# Autodesk Inventor assembly: Frame
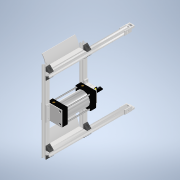
[picture p0: Inventor's stored thumbnail of the model, 180x180]
Saved by Autodesk Inventor 2022 (Build 260153000, 153)
## iProperties
Created: 2022-02-15
Part Number: Frame
Document SubType Name: Assembly
Designer: siwat
Author: siwat
## Documents named in this file (10)
- D:\Git\osu-cbt\CAD\Frame\Frame.iam
- D:\Git\osu-cbt\CAD\Frame\Aluminium_VSlot_40cm.ipt
- D:\Git\osu-cbt\CAD\Frame\OpenBuilds\Black Angle Corner Connector.ipt
- D:\Git\osu-cbt\CAD\Frame\SC63X100-S.ipt
- D:\Git\osu-cbt\CAD\Frame\FrontPistonSupportButtom.ipt
- D:\Git\osu-cbt\CAD\Frame\FrontPistonSupportTop.ipt
- D:\Git\osu-cbt\CAD\Frame\BackPistonSupport Top.ipt
- D:\Git\osu-cbt\CAD\Frame\Prototype 2\BackPistonSupportButtom.ipt
- D:\Git\osu-cbt\CAD\Frame\LegSupport.ipt
- D:\Git\osu-cbt\CAD\Frame\StrapHolder.ipt
## Components (21 placed, 10 different names)
1. 40cm_V-Slot — Flush:1, Mate:1, Flush:2, Mate:2, Flush:3, Flush:4, Mate:6, Flush:9, Mate:8, Flush:10, Mate:10, Flush:11, Mate:11, Flush:12, Mate:19, Mate:20
2. Black Angle Corner Connector:1 — Mate:2, Flush:3, Flush:4, Mate:5
3. Black Angle Corner Connector:4 — Flush:1, Mate:1, Flush:2, Mate:9
4. Aluminium_VSlot_40cm:3 — Mate:5, Mate:6, Flush:9, Mate:7, Mate:17, Mate:18, Mate:22, Mate:23, Flush:27, Mate:27, Mate:28, Flush:32, Mate:30
5. Black Angle Corner Connector:5 — Mate:11, Mate:12, Flush:12
6. Black Angle Corner Connector:6 — Mate:7, Mate:8, Flush:10
7. Aluminium_VSlot_40cm:4 — Mate:9, Mate:10, Flush:11, Mate:12, Mate:25, Flush:28, Flush:29, Flush:30, Flush:31, Mate:29
8. Aluminium_VSlot_40cm:5 — Mate:18, Mate:21, Flush:19, Flush:20, Mate:24, Mate:26
9. Black Angle Corner Connector:7 — Mate:17
10. Black Angle Corner Connector:8
11. Black Angle Corner Connector:9 — Mate:29
12. Black Angle Corner Connector:10 — Mate:30
13. SC63X100-S:1 — Mate:19, Mate:20, Mate:21, Mate:22, Flush:23, Flush:24, Flush:25, Flush:26
14. FrontPistonSupportButtom:1 — Flush:19, Flush:20, Flush:21, Flush:22, Flush:33
15. FrontPistonSupportTop:1 — Flush:21, Flush:22, Flush:33
16. BackPistonSupport Top:1 — Flush:23, Flush:24
17. BackPistonSupportButtom:1 — Flush:25, Flush:26
18. LegSupport:1 — Mate:23, Flush:27, Mate:24
19. LegSupport:2 — Mate:25, Mate:26, Flush:28
20. StrapHolder:1 — Flush:29, Flush:30, Flush:31
21. StrapHolder:2 — Mate:27, Mate:28, Flush:32
## Relationships (57: Flush 29, Mate 28)
- Flush:1: 40cm_V-Slot ↔ Black Angle Corner Connector:4
- Mate:1: 40cm_V-Slot ↔ Black Angle Corner Connector:4
- Flush:2: 40cm_V-Slot ↔ Black Angle Corner Connector:4
- Mate:2: 40cm_V-Slot ↔ Black Angle Corner Connector:1
- Flush:3: 40cm_V-Slot ↔ Black Angle Corner Connector:1
- Flush:4: 40cm_V-Slot ↔ Black Angle Corner Connector:1
- Mate:5: Black Angle Corner Connector:1 ↔ Aluminium_VSlot_40cm:3
- Mate:6: 40cm_V-Slot ↔ Aluminium_VSlot_40cm:3
- Flush:9: 40cm_V-Slot ↔ Aluminium_VSlot_40cm:3
- Mate:7: Aluminium_VSlot_40cm:3 ↔ Black Angle Corner Connector:6
- Mate:8: 40cm_V-Slot ↔ Black Angle Corner Connector:6
- Flush:10: 40cm_V-Slot ↔ Black Angle Corner Connector:6
- Mate:9: Black Angle Corner Connector:4 ↔ Aluminium_VSlot_40cm:4
- Mate:10: 40cm_V-Slot ↔ Aluminium_VSlot_40cm:4
- Flush:11: 40cm_V-Slot ↔ Aluminium_VSlot_40cm:4
- Mate:11: 40cm_V-Slot ↔ Black Angle Corner Connector:5
- Mate:12: Black Angle Corner Connector:5 ↔ Aluminium_VSlot_40cm:4
- Flush:12: 40cm_V-Slot ↔ Black Angle Corner Connector:5
- [Flush]: Aluminium_VSlot_40cm:5 ↔ Black Angle Corner Connector:8
- [Mate]: Aluminium_VSlot_40cm:5 ↔ Black Angle Corner Connector:8
- [Flush]: Aluminium_VSlot_40cm:5 ↔ Black Angle Corner Connector:8
- [Mate]: Aluminium_VSlot_40cm:5 ↔ Black Angle Corner Connector:7
- [Flush]: Aluminium_VSlot_40cm:5 ↔ Black Angle Corner Connector:7
- [Flush]: Aluminium_VSlot_40cm:5 ↔ Black Angle Corner Connector:7
- [Mate]: Aluminium_VSlot_40cm:5 ↔ Black Angle Corner Connector:10
- [Flush]: Aluminium_VSlot_40cm:5 ↔ Black Angle Corner Connector:10
- [Mate]: Aluminium_VSlot_40cm:5 ↔ Black Angle Corner Connector:9
- [Flush]: Aluminium_VSlot_40cm:5 ↔ Black Angle Corner Connector:9
- Mate:17: Aluminium_VSlot_40cm:3 ↔ Black Angle Corner Connector:7
- Mate:18: Aluminium_VSlot_40cm:3 ↔ Aluminium_VSlot_40cm:5
- Mate:19: 40cm_V-Slot ↔ SC63X100-S:1
- Mate:20 (-12 mm): 40cm_V-Slot ↔ SC63X100-S:1
- Mate:21: Aluminium_VSlot_40cm:5 ↔ SC63X100-S:1
- Mate:22 (125 mm): Aluminium_VSlot_40cm:3 ↔ SC63X100-S:1
- Flush:19: Aluminium_VSlot_40cm:5 ↔ FrontPistonSupportButtom:1
- Flush:20: Aluminium_VSlot_40cm:5 ↔ FrontPistonSupportButtom:1
- Flush:21: FrontPistonSupportButtom:1 ↔ FrontPistonSupportTop:1
- Flush:22: FrontPistonSupportButtom:1 ↔ FrontPistonSupportTop:1
- Flush:23: SC63X100-S:1 ↔ BackPistonSupport Top:1
- Flush:24: SC63X100-S:1 ↔ BackPistonSupport Top:1
- Flush:25: SC63X100-S:1 ↔ BackPistonSupportButtom:1
- Flush:26: SC63X100-S:1 ↔ BackPistonSupportButtom:1
- Mate:23: Aluminium_VSlot_40cm:3 ↔ LegSupport:1
- Flush:27: Aluminium_VSlot_40cm:3 ↔ LegSupport:1
- Mate:24: Aluminium_VSlot_40cm:5 ↔ LegSupport:1
- Mate:25: Aluminium_VSlot_40cm:4 ↔ LegSupport:2
- Mate:26: Aluminium_VSlot_40cm:5 ↔ LegSupport:2
- Flush:28: Aluminium_VSlot_40cm:4 ↔ LegSupport:2
- Flush:29: Aluminium_VSlot_40cm:4 ↔ StrapHolder:1
- Flush:30: Aluminium_VSlot_40cm:4 ↔ StrapHolder:1
- Flush:31: Aluminium_VSlot_40cm:4 ↔ StrapHolder:1
- Mate:27: Aluminium_VSlot_40cm:3 ↔ StrapHolder:2
- Mate:28: Aluminium_VSlot_40cm:3 ↔ StrapHolder:2
- Flush:32: Aluminium_VSlot_40cm:3 ↔ StrapHolder:2
- Mate:29: Aluminium_VSlot_40cm:4 ↔ Black Angle Corner Connector:9
- Mate:30: Aluminium_VSlot_40cm:3 ↔ Black Angle Corner Connector:10
- Flush:33: FrontPistonSupportButtom:1 ↔ FrontPistonSupportTop:1
## Named parameters: d26_d0 = 0 mm, d27_d19 = 0 mm, d28_d23 = 0 mm, d29_d25 = 0 mm, d30_d18 = 0 mm, d31_d1 = 0 mm, d32_d2 = 0 mm, d33_d3 = 0 mm, d34_d4 = 0 mm, d35_d5 = 0 mm
